# Autodesk Inventor assembly: invacare assy
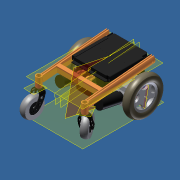
[picture p0: Inventor's stored thumbnail of the model, 180x180]
Saved by Autodesk Inventor 2012 (Build 160160000, 160)
## iProperties
Created: 2012-03-08
Part Number: invacare assy
Document SubType Name: Assembly
Designer: esv
Mass: 83979.9 g
Surface Area: 24308.3 cm^2
Volume: 48170.3 cm^3
Density: 1.7434 g/cm^3
Author: esv
## Documents named in this file (5)
- C:\Users\Edward\Documents\masters\CAD\Invacare\invacare assy.iam
- C:\Users\Edward\Documents\masters\CAD\Invacare\wheel.ipt
- C:\Users\Edward\Documents\masters\CAD\Invacare\frame_solid.iam
- C:\Users\Edward\Documents\masters\CAD\Invacare\caster wheel.ipt
- C:\Users\Edward\Documents\masters\CAD\Invacare\caster.ipt
## Components (7 placed, 7 different names)
1. frame_solid:1 [sub-assembly] — Insert:3, Insert:4, Insert:7, Insert:8
2. l_drive_wheel — Insert:3
3. r_drive wheel — Insert:4
4. r_caster_wheel — Insert:5
5. r_caster — Insert:5, Insert:8
6. l_caster_wheel — Insert:6
7. l_caster — Insert:6, Insert:7
## Relationships (6: Insert 6)
- Insert:3: frame_solid:1 ↔ l_drive_wheel
- Insert:4: frame_solid:1 ↔ r_drive wheel
- Insert:5: r_caster_wheel ↔ r_caster
- Insert:6: l_caster_wheel ↔ l_caster
- Insert:7: frame_solid:1 ↔ l_caster
- Insert:8: frame_solid:1 ↔ r_caster
